# Autodesk Inventor assembly: 00_XY_stage-CHUO_SEIKI_LD-647-R1
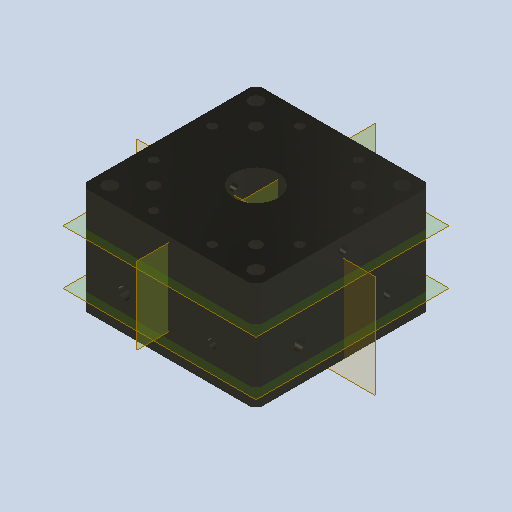
[picture p0: Inventor's stored thumbnail of the model, 512x512]
Saved by Autodesk Inventor 2022.3 (Build 263350000, 350)
## iProperties
Created: 2019-05-02
Part Number: 00_XY_stage-CHUO_SEIKI_LD-647-R1
Document SubType Name: Assembly
Designer: diederichbenedict
Author: diederichbenedict
## Documents named in this file (4)
- G:\My Drive\ASP - M.Sc. Photonics\Practical Modules\MODULE 4 - Master Thesis\2.Experiments\Modules\13.XY_Stage_with_Cubes\00_XY_stage-CHUO_SEIKI_LD-647-R1.iam
- G:\My Drive\ASP - M.Sc. Photonics\Practical Modules\MODULE 4 - Master Thesis\2.Experiments\Modules\13.XY_Stage_with_Cubes\00_XY_stage-CHUO_SEIKI_LD-647-R1-Top.ipt
- G:\My Drive\ASP - M.Sc. Photonics\Practical Modules\MODULE 4 - Master Thesis\2.Experiments\Modules\13.XY_Stage_with_Cubes\00_XY_stage-CHUO_SEIKI_LD-647-R1-Middle.ipt
- G:\My Drive\ASP - M.Sc. Photonics\Practical Modules\MODULE 4 - Master Thesis\2.Experiments\Modules\13.XY_Stage_with_Cubes\00_XY_stage-CHUO_SEIKI_LD-647-R1-Bottom.ipt
## Components (3 placed, 3 different names)
1. 00_XY_stage-CHUO_SEIKI_LD-647-R1-Top:1 — Flush:1, Flush:2, Mate:1, Symmetry:1, Symmetry:2
2. 00_XY_stage-CHUO_SEIKI_LD-647-R1-Middle:1 — Flush:1, Flush:2, Flush:3, Flush:4, Mate:1, Symmetry:1, Symmetry:2, Symmetry:3
3. 00_XY_stage-CHUO_SEIKI_LD-647-R1-Bottom:1 — Flush:3, Flush:4, Symmetry:3
## Relationships (8: Flush 4, Symmetry 3, Mate 1)
- Flush:1: 00_XY_stage-CHUO_SEIKI_LD-647-R1-Top:1 ↔ 00_XY_stage-CHUO_SEIKI_LD-647-R1-Middle:1
- Flush:2: 00_XY_stage-CHUO_SEIKI_LD-647-R1-Top:1 ↔ 00_XY_stage-CHUO_SEIKI_LD-647-R1-Middle:1
- Flush:3: 00_XY_stage-CHUO_SEIKI_LD-647-R1-Middle:1 ↔ 00_XY_stage-CHUO_SEIKI_LD-647-R1-Bottom:1
- Flush:4: 00_XY_stage-CHUO_SEIKI_LD-647-R1-Middle:1 ↔ 00_XY_stage-CHUO_SEIKI_LD-647-R1-Bottom:1
- Mate:1: 00_XY_stage-CHUO_SEIKI_LD-647-R1-Top:1 ↔ 00_XY_stage-CHUO_SEIKI_LD-647-R1-Middle:1
- Symmetry:1: 00_XY_stage-CHUO_SEIKI_LD-647-R1-Top:1 ↔ 00_XY_stage-CHUO_SEIKI_LD-647-R1-Middle:1
- Symmetry:2: 00_XY_stage-CHUO_SEIKI_LD-647-R1-Top:1 ↔ 00_XY_stage-CHUO_SEIKI_LD-647-R1-Middle:1
- Symmetry:3: 00_XY_stage-CHUO_SEIKI_LD-647-R1-Middle:1 ↔ 00_XY_stage-CHUO_SEIKI_LD-647-R1-Bottom:1
